# Autodesk Inventor assembly: gyroPhone06
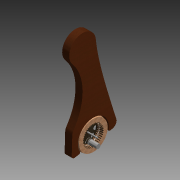
[picture p0: Inventor's stored thumbnail of the model, 180x180]
Saved by Autodesk Inventor 2013 (Build 170138000, 138)
## iProperties
Created: 2013-01-21
Part Number: gyroPhone06
Document SubType Name: Assembly
Designer: Nano
Author: Nano
## Documents named in this file (4)
- C:\Users\Nano\Documents\InventorByron\InventorMasterProject\gyroPhone01\gyroPhone06.iam
- C:\Users\Nano\Documents\InventorByron\InventorMasterProject\gyroPhone01\wheelAssembly01.iam
- C:\Users\Nano\Documents\InventorByron\InventorMasterProject\gyroPhone01\motorDriveWheelAssembly.iam
- C:\Users\Nano\Documents\InventorByron\InventorMasterProject\gyroPhone01\body01.ipt
## Components (3 placed, 3 different names)
1. wheelAssembly01:1 [sub-assembly] — Mate:1, Mate:2, Flush:2
2. motorDriveWheelAssembly:1 [sub-assembly] — Mate:1, Mate:2
3. body01:1 — Flush:1, Flush:2
## Relationships (4: Mate 2, Flush 2)
- Mate:1 (3.175 mm): wheelAssembly01:1 ↔ motorDriveWheelAssembly:1
- Mate:2: wheelAssembly01:1 ↔ motorDriveWheelAssembly:1
- Flush:1: body01:1
- Flush:2: wheelAssembly01:1 ↔ body01:1
